# Autodesk Inventor assembly: Plasma-flange-support
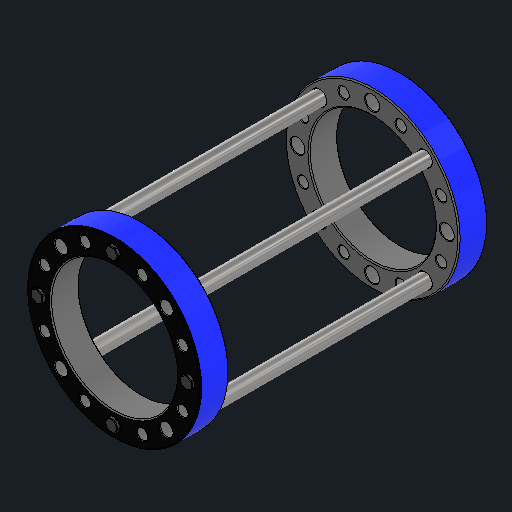
[picture p0: Inventor's stored thumbnail of the model, 512x512]
Saved by Autodesk Inventor 2025 (Build 290162000, 162)
## iProperties
Created: 2024-05-24
Part Number: Plasma-flange-support
Document SubType Name: Assembly
Designer: kuzmin
Author: kuzmin
## Documents named in this file (5)
- C:\Users\queezz\Dropbox\Drawings\PIHTI\Scaffolding\Plasma-flange-support.iam
- C:\Users\queezz\Dropbox\Drawings\PIHTI\Scaffolding\CF150-spacer.ipt
- C:\Users\queezz\Dropbox\Drawings\PIHTI\Scaffolding\Rod-12x220-M6.ipt
- C:\Users\queezz\Dropbox\Drawings\PIHTI\ContentCenter\Fastners\M6x25-SHCS.ipt
- C:\Users\queezz\Dropbox\Drawings\PIHTI\Scaffolding\TPU-legs.ipt
## Components (14 placed, 4 different names)
1. CF150-spacer:1 — Rigid:14, Rigid:15, Rigid:16, Rigid:17, Rigid:18, Rigid:19, Rigid:20, Rigid:21
2. CF150-spacer:2 — Rotational:6, Rigid:10, Rigid:11, Rigid:12, Rigid:13, Mate:1
3. Rod-12x220-M6:1 — Rotational:6, Rigid:17
4. Rod-12x220-M6:2 — Rigid:16
5. Rod-12x220-M6:3 — Rigid:14
6. Rod-12x220-M6:4 — Rigid:15, Mate:1
7. TPU-legs:1 — Rigid:19
8. TPU-legs:2 — Rigid:18
9. TPU-legs:3 — Rigid:20
10. TPU-legs:4 — Rigid:21
11. IS 2269 M6 x 25:1 — Rigid:10
12. IS 2269 M6 x 25:2 — Rigid:11
13. IS 2269 M6 x 25:3 — Rigid:12
14. IS 2269 M6 x 25:4 — Rigid:13
## Relationships (14: WeldJoint 12, RevoluteJoint 1, Mate 1)
- Rotational:6 [RevoluteJoint]: CF150-spacer:2 ↔ Rod-12x220-M6:1
- Rigid:10 [WeldJoint]: CF150-spacer:2 ↔ IS 2269 M6 x 25:1
- Rigid:11 [WeldJoint]: CF150-spacer:2 ↔ IS 2269 M6 x 25:2
- Rigid:12 [WeldJoint]: CF150-spacer:2 ↔ IS 2269 M6 x 25:3
- Rigid:13 [WeldJoint]: CF150-spacer:2 ↔ IS 2269 M6 x 25:4
- Rigid:14 [WeldJoint]: CF150-spacer:1 ↔ Rod-12x220-M6:3
- Rigid:15 [WeldJoint]: CF150-spacer:1 ↔ Rod-12x220-M6:4
- Rigid:16 [WeldJoint]: CF150-spacer:1 ↔ Rod-12x220-M6:2
- Rigid:17 [WeldJoint]: CF150-spacer:1 ↔ Rod-12x220-M6:1
- Mate:1: CF150-spacer:2 ↔ Rod-12x220-M6:4
- Rigid:18 [WeldJoint]: CF150-spacer:1 ↔ TPU-legs:2
- Rigid:19 [WeldJoint]: CF150-spacer:1 ↔ TPU-legs:1
- Rigid:20 [WeldJoint]: CF150-spacer:1 ↔ TPU-legs:3
- Rigid:21 [WeldJoint]: CF150-spacer:1 ↔ TPU-legs:4
